# Autodesk Inventor assembly: 4-bar assembly 2
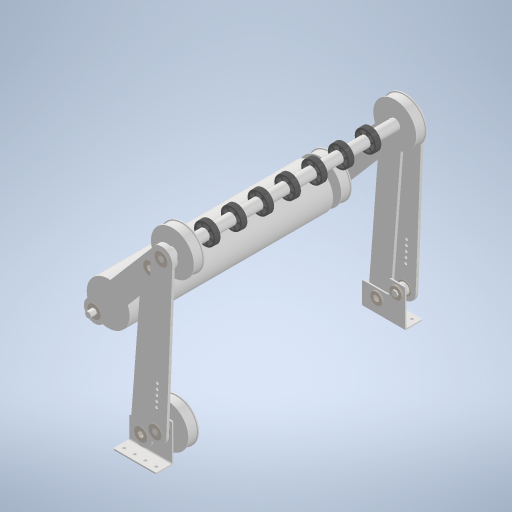
[picture p0: Inventor's stored thumbnail of the model, 512x512]
Saved by Autodesk Inventor 2023 (Build 270158030, 158C)
## iProperties
Created: 2022-07-19
Part Number: 4-bar assembly 2
Document SubType Name: Assembly
Designer: rm0990889
Author: rm0990889
## Documents named in this file (16)
- C:\Users\rm0990889\Downloads\FIRST CAD-20220720T142030Z-001\FIRST CAD\4-bar intake practice-20220720T134858Z-001\4-bar intake practice\4-bar assembly 2.iam
- C:\Users\rm0990889\Downloads\FIRST CAD-20220720T142030Z-001\FIRST CAD\4-bar intake practice-20220720T134858Z-001\4-bar intake practice\4-bar intake mount.ipt
- C:\Users\rm0990889\Downloads\FIRST CAD-20220720T142030Z-001\FIRST CAD\4-bar intake practice-20220720T134858Z-001\4-bar intake practice\4-bar intake (14.112) bar.ipt
- C:\Users\rm0990889\Downloads\FIRST CAD-20220720T142030Z-001\FIRST CAD\4-bar intake practice-20220720T134858Z-001\4-bar intake practice\am-2986 FR8ZZ Hex Bearing.ipt
- C:\Users\rm0990889\Downloads\FIRST CAD-20220720T142030Z-001\FIRST CAD\4-bar intake practice-20220720T134858Z-001\4-bar intake practice\4-bar intake spacer.ipt
- C:\Users\rm0990889\Downloads\FIRST CAD-20220720T142030Z-001\FIRST CAD\4-bar intake practice-20220720T134858Z-001\4-bar intake practice\4-bar intake (14.258) bar.ipt
- C:\Users\rm0990889\Downloads\FIRST CAD-20220720T142030Z-001\FIRST CAD\4-bar intake practice-20220720T134858Z-001\4-bar intake practice\4-bar intake (24) shaft.ipt
- C:\Users\rm0990889\Downloads\FIRST CAD-20220720T142030Z-001\FIRST CAD\4-bar intake practice-20220720T134858Z-001\4-bar intake practice\4-bar intake peg.ipt
- C:\Users\rm0990889\Downloads\FIRST CAD-20220720T142030Z-001\FIRST CAD\4-bar intake practice-20220720T134858Z-001\4-bar intake practice\4-bar intake (2) shaft.ipt
- C:\Users\rm0990889\Downloads\FIRST CAD-20220720T142030Z-001\FIRST CAD\4-bar intake practice-20220720T134858Z-001\4-bar intake practice\4-bar intake () pully.ipt
- C:\Users\rm0990889\Downloads\FIRST CAD-20220720T142030Z-001\FIRST CAD\4-bar intake practice-20220720T134858Z-001\4-bar intake practice\am-3462 2IN Molded 500Hex Compliant Wheel REV2.ipt
- C:\Users\rm0990889\Downloads\FIRST CAD-20220720T142030Z-001\FIRST CAD\4-bar intake practice-20220720T134858Z-001\4-bar intake practice\4-bar intake (2_) spacer.ipt
- C:\Users\rm0990889\Downloads\FIRST CAD-20220720T142030Z-001\FIRST CAD\4-bar intake practice-20220720T134858Z-001\4-bar intake practice\4-bar intake block.ipt
- C:\Users\rm0990889\Downloads\FIRST CAD-20220720T142030Z-001\FIRST CAD\4-bar intake practice-20220720T134858Z-001\4-bar intake practice\4-bar intake roller.ipt
- C:\Users\rm0990889\Downloads\FIRST CAD-20220720T142030Z-001\FIRST CAD\4-bar intake practice-20220720T134858Z-001\4-bar intake practice\4-bar intake (1_) spacer.ipt
- C:\Users\rm0990889\Downloads\FIRST CAD-20220720T142030Z-001\FIRST CAD\4-bar intake practice-20220720T134858Z-001\4-bar intake practice\4-bar intake mount(alt).ipt
## Components (63 placed, 15 different names)
1. 4-bar intake mount:1 — Insert:1, Insert:2, Flush:3, Flush:4
2. 4-bar intake (14.112) bar:1 — Insert:3, Insert:4
3. am-2986 FR8ZZ Hex Bearing:1 — Insert:1, Insert:5
4. am-2986 FR8ZZ Hex Bearing:2 — Insert:2, Insert:6, Insert:11
5. am-2986 FR8ZZ Hex Bearing:3 — Insert:3, Insert:5
6. am-2986 FR8ZZ Hex Bearing:4 — Insert:4, Mate:33
7. am-2986 FR8ZZ Hex Bearing:5 — Insert:8, Insert:10, Mate:7
8. am-2986 FR8ZZ Hex Bearing:6 — Insert:19, Mate:37, Mate:38, Insert:45
9. am-2986 FR8ZZ Hex Bearing:7 — Insert:9, Mate:1, Mate:2
10. am-2986 FR8ZZ Hex Bearing:8 — Insert:21, Mate:50
11. am-2986 FR8ZZ Hex Bearing:9 — Insert:20, Mate:33
12. am-2986 FR8ZZ Hex Bearing:10 — Insert:22, Mate:54, Mate:55
13. am-2986 FR8ZZ Hex Bearing:11 — Insert:24, Flush:2, Mate:51, Mate:53
14. am-2986 FR8ZZ Hex Bearing:12 — Insert:23, Mate:49
15. am-2986 FR8ZZ Hex Bearing:13 — Insert:49, Insert:56
16. am-2986 FR8ZZ Hex Bearing:14 — Insert:50, Insert:55
17. 4-bar intake spacer:2 — Mate:9, Insert:14, Mate:50
18. 4-bar intake spacer:3 — Insert:14, Mate:10, Insert:15, Insert:26
19. 4-bar intake spacer:4 — Insert:6, Insert:7
20. 4-bar intake spacer:5 — Insert:35, Insert:62
21. 4-bar intake spacer:6 — Insert:7, Insert:10
22. 4-bar intake (14.258) bar:1 — Insert:8, Insert:9, Insert:25
23. 4-bar intake (24) shaft:1 — Mate:37, Mate:38, Mate:39, Mate:40, Mate:54, Mate:55
24. 4-bar intake (24) shaft:2 — Mate:1, Mate:2, Mate:9, Mate:10, Mate:11, Mate:30, Mate:31, Mate:32, Mate:34, Mate:35, Mate:36, Mate:41, Mate:42, Mate:43, Mate:44, Mate:51, Mate:52
25. 4-bar intake peg:1 — Mate:47, Mate:48, Flush:1
26. 4-bar intake (2) shaft:2 — Mate:5, Mate:6, Mate:7
27. 4-bar intake () pully:1 — Mate:5, Mate:6, Insert:11
28. 4-bar intake () pully:2 — Insert:15, Mate:11, Insert:26, Mate:30, Mate:31, Insert:27
29. am-3462 2IN Molded 500Hex Compliant Wheel REV2:8 — Insert:34, Insert:37
30. am-3462 2IN Molded 500Hex Compliant Wheel REV2:9 — Insert:32, Insert:33
31. am-3462 2IN Molded 500Hex Compliant Wheel REV2:10 — Insert:30, Insert:31
32. am-3462 2IN Molded 500Hex Compliant Wheel REV2:11 — Insert:28, Insert:29
33. 4-bar intake block:1 — Insert:22, Insert:23, Insert:24, Insert:59
34. 4-bar intake block:2 — Insert:19, Insert:20, Insert:21, Insert:25
35. 4-bar intake (2_) spacer:8 — Insert:37, Mate:41, Insert:38
36. 4-bar intake (2_) spacer:9 — Insert:33, Mate:36, Insert:34
37. 4-bar intake (2_) spacer:11 — Insert:27, Mate:32, Insert:28
38. 4-bar intake (2_) spacer:12 — Insert:29, Mate:34, Insert:30
39. 4-bar intake (2_) spacer:13 — Insert:31, Mate:35, Insert:32
40. 4-bar intake roller:1 — Mate:39, Mate:40, Insert:35, Insert:46
41. am-3462 2IN Molded 500Hex Compliant Wheel REV2:12 — Insert:38, Insert:39
42. am-3462 2IN Molded 500Hex Compliant Wheel REV2:13 — Insert:40, Insert:41
43. am-3462 2IN Molded 500Hex Compliant Wheel REV2:15 — Insert:42, Insert:43
44. 4-bar intake (2_) spacer:15 — Insert:39, Mate:42, Insert:40
45. 4-bar intake (2_) spacer:16 — Insert:41, Mate:43, Insert:42
46. 4-bar intake (2_) spacer:17 — Insert:43, Mate:44, Insert:47
47. 4-bar intake (1_) spacer:1 — Insert:45, Insert:46
48. 4-bar intake spacer:7 — Insert:47, Insert:48
49. 4-bar intake () pully:4 — Insert:48, Insert:61
50. 4-bar intake mount(alt):1 — Insert:49, Insert:50, Flush:3, Flush:4
51. 4-bar intake (14.112) bar:2 — Insert:51, Insert:52, Insert:55
52. 4-bar intake (14.258) bar:2 — Insert:53, Insert:54, Insert:59
53. am-2986 FR8ZZ Hex Bearing:15 — Insert:52, Mate:49
54. am-2986 FR8ZZ Hex Bearing:16 — Insert:54, Insert:58, Mate:47, Mate:48, Flush:1
55. am-2986 FR8ZZ Hex Bearing:17 — Insert:51
56. am-2986 FR8ZZ Hex Bearing:18 — Insert:53, Flush:2, Mate:52
57. 4-bar intake spacer:8 — Insert:56, Insert:57
58. 4-bar intake spacer:9 — Insert:57, Insert:58
59. 4-bar intake spacer:11 — Insert:61, Mate:53
60. 4-bar intake spacer:12 — Insert:63, Insert:64
61. 4-bar intake spacer:14 — Insert:65
62. 4-bar intake spacer:15 — Insert:62, Insert:63
63. 4-bar intake () pully:5 — Insert:64, Insert:65
## Relationships (93: Insert 57, Mate 32, Flush 4)
- Insert:1: 4-bar intake mount:1 ↔ am-2986 FR8ZZ Hex Bearing:1
- Insert:2: 4-bar intake mount:1 ↔ am-2986 FR8ZZ Hex Bearing:2
- Insert:3: 4-bar intake (14.112) bar:1 ↔ am-2986 FR8ZZ Hex Bearing:3
- Insert:4: 4-bar intake (14.112) bar:1 ↔ am-2986 FR8ZZ Hex Bearing:4
- Insert:5: am-2986 FR8ZZ Hex Bearing:1 ↔ am-2986 FR8ZZ Hex Bearing:3
- Insert:6: am-2986 FR8ZZ Hex Bearing:2 ↔ 4-bar intake spacer:4
- Insert:7: 4-bar intake spacer:4 ↔ 4-bar intake spacer:6
- Insert:8: am-2986 FR8ZZ Hex Bearing:5 ↔ 4-bar intake (14.258) bar:1
- Insert:9: am-2986 FR8ZZ Hex Bearing:7 ↔ 4-bar intake (14.258) bar:1
- Insert:10: am-2986 FR8ZZ Hex Bearing:5 ↔ 4-bar intake spacer:6
- Mate:1: am-2986 FR8ZZ Hex Bearing:7 ↔ 4-bar intake (24) shaft:2
- Mate:2: am-2986 FR8ZZ Hex Bearing:7 ↔ 4-bar intake (24) shaft:2
- Mate:5: 4-bar intake (2) shaft:2 ↔ 4-bar intake () pully:1
- Mate:6: 4-bar intake (2) shaft:2 ↔ 4-bar intake () pully:1
- Insert:11: am-2986 FR8ZZ Hex Bearing:2 ↔ 4-bar intake () pully:1
- Mate:7: am-2986 FR8ZZ Hex Bearing:5 ↔ 4-bar intake (2) shaft:2
- Mate:9: 4-bar intake spacer:2 ↔ 4-bar intake (24) shaft:2
- Insert:14: 4-bar intake spacer:2 ↔ 4-bar intake spacer:3
- Mate:10: 4-bar intake spacer:3 ↔ 4-bar intake (24) shaft:2
- Insert:15: 4-bar intake spacer:3 ↔ 4-bar intake () pully:2
- Mate:11: 4-bar intake (24) shaft:2 ↔ 4-bar intake () pully:2
- Insert:19: am-2986 FR8ZZ Hex Bearing:6 ↔ 4-bar intake block:2
- Insert:20: am-2986 FR8ZZ Hex Bearing:9 ↔ 4-bar intake block:2
- Insert:21: am-2986 FR8ZZ Hex Bearing:8 ↔ 4-bar intake block:2
- Insert:22: am-2986 FR8ZZ Hex Bearing:10 ↔ 4-bar intake block:1
- Insert:23: am-2986 FR8ZZ Hex Bearing:12 ↔ 4-bar intake block:1
- Insert:24: am-2986 FR8ZZ Hex Bearing:11 ↔ 4-bar intake block:1
- Insert:25: 4-bar intake (14.258) bar:1 ↔ 4-bar intake block:2
- Insert:26: 4-bar intake spacer:3 ↔ 4-bar intake () pully:2
- Mate:30: 4-bar intake (24) shaft:2 ↔ 4-bar intake () pully:2
- Mate:31: 4-bar intake (24) shaft:2 ↔ 4-bar intake () pully:2
- Insert:27: 4-bar intake () pully:2 ↔ 4-bar intake (2_) spacer:11
- Mate:32: 4-bar intake (24) shaft:2 ↔ 4-bar intake (2_) spacer:11
- Insert:28: am-3462 2IN Molded 500Hex Compliant Wheel REV2:11 ↔ 4-bar intake (2_) spacer:11
- Mate:33: am-2986 FR8ZZ Hex Bearing:4 ↔ am-2986 FR8ZZ Hex Bearing:9
- Insert:29: am-3462 2IN Molded 500Hex Compliant Wheel REV2:11 ↔ 4-bar intake (2_) spacer:12
- Mate:34: 4-bar intake (24) shaft:2 ↔ 4-bar intake (2_) spacer:12
- Insert:30: am-3462 2IN Molded 500Hex Compliant Wheel REV2:10 ↔ 4-bar intake (2_) spacer:12
- Insert:31: am-3462 2IN Molded 500Hex Compliant Wheel REV2:10 ↔ 4-bar intake (2_) spacer:13
- Mate:35: 4-bar intake (24) shaft:2 ↔ 4-bar intake (2_) spacer:13
- Insert:32: am-3462 2IN Molded 500Hex Compliant Wheel REV2:9 ↔ 4-bar intake (2_) spacer:13
- Insert:33: am-3462 2IN Molded 500Hex Compliant Wheel REV2:9 ↔ 4-bar intake (2_) spacer:9
- Mate:36: 4-bar intake (24) shaft:2 ↔ 4-bar intake (2_) spacer:9
- Insert:34: am-3462 2IN Molded 500Hex Compliant Wheel REV2:8 ↔ 4-bar intake (2_) spacer:9
- Mate:37: am-2986 FR8ZZ Hex Bearing:6 ↔ 4-bar intake (24) shaft:1
- Mate:38: am-2986 FR8ZZ Hex Bearing:6 ↔ 4-bar intake (24) shaft:1
- Mate:39: 4-bar intake (24) shaft:1 ↔ 4-bar intake roller:1
- Mate:40: 4-bar intake (24) shaft:1 ↔ 4-bar intake roller:1
- Insert:35: 4-bar intake spacer:5 ↔ 4-bar intake roller:1
- Insert:37: am-3462 2IN Molded 500Hex Compliant Wheel REV2:8 ↔ 4-bar intake (2_) spacer:8
- Mate:41: 4-bar intake (24) shaft:2 ↔ 4-bar intake (2_) spacer:8
- Insert:38: 4-bar intake (2_) spacer:8 ↔ am-3462 2IN Molded 500Hex Compliant Wheel REV2:12
- Insert:39: am-3462 2IN Molded 500Hex Compliant Wheel REV2:12 ↔ 4-bar intake (2_) spacer:15
- Mate:42: 4-bar intake (24) shaft:2 ↔ 4-bar intake (2_) spacer:15
- Insert:40: am-3462 2IN Molded 500Hex Compliant Wheel REV2:13 ↔ 4-bar intake (2_) spacer:15
- Insert:41: am-3462 2IN Molded 500Hex Compliant Wheel REV2:13 ↔ 4-bar intake (2_) spacer:16
- Mate:43: 4-bar intake (24) shaft:2 ↔ 4-bar intake (2_) spacer:16
- Insert:42: am-3462 2IN Molded 500Hex Compliant Wheel REV2:15 ↔ 4-bar intake (2_) spacer:16
- Insert:43: am-3462 2IN Molded 500Hex Compliant Wheel REV2:15 ↔ 4-bar intake (2_) spacer:17
- Mate:44: 4-bar intake (24) shaft:2 ↔ 4-bar intake (2_) spacer:17
- Insert:45: am-2986 FR8ZZ Hex Bearing:6 ↔ 4-bar intake (1_) spacer:1
- Insert:46: 4-bar intake roller:1 ↔ 4-bar intake (1_) spacer:1
- Insert:47: 4-bar intake (2_) spacer:17 ↔ 4-bar intake spacer:7
- Insert:48: 4-bar intake spacer:7 ↔ 4-bar intake () pully:4
- Insert:49: am-2986 FR8ZZ Hex Bearing:13 ↔ 4-bar intake mount(alt):1
- Insert:50: am-2986 FR8ZZ Hex Bearing:14 ↔ 4-bar intake mount(alt):1
- Insert:51: 4-bar intake (14.112) bar:2 ↔ am-2986 FR8ZZ Hex Bearing:17
- Insert:52: 4-bar intake (14.112) bar:2 ↔ am-2986 FR8ZZ Hex Bearing:15
- Insert:53: 4-bar intake (14.258) bar:2 ↔ am-2986 FR8ZZ Hex Bearing:18
- Insert:54: 4-bar intake (14.258) bar:2 ↔ am-2986 FR8ZZ Hex Bearing:16
- Insert:55: am-2986 FR8ZZ Hex Bearing:14 ↔ 4-bar intake (14.112) bar:2
- Insert:56: am-2986 FR8ZZ Hex Bearing:13 ↔ 4-bar intake spacer:8
- Insert:57: 4-bar intake spacer:8 ↔ 4-bar intake spacer:9
- Insert:58: am-2986 FR8ZZ Hex Bearing:16 ↔ 4-bar intake spacer:9
- Mate:47: 4-bar intake peg:1 ↔ am-2986 FR8ZZ Hex Bearing:16
- Mate:48: 4-bar intake peg:1 ↔ am-2986 FR8ZZ Hex Bearing:16
- Flush:1: 4-bar intake peg:1 ↔ am-2986 FR8ZZ Hex Bearing:16
- Insert:59: 4-bar intake block:1 ↔ 4-bar intake (14.258) bar:2
- Mate:49: am-2986 FR8ZZ Hex Bearing:12 ↔ am-2986 FR8ZZ Hex Bearing:15
- Insert:61: 4-bar intake () pully:4 ↔ 4-bar intake spacer:11
- Mate:50: am-2986 FR8ZZ Hex Bearing:8 ↔ 4-bar intake spacer:2
- Insert:62: 4-bar intake spacer:5 ↔ 4-bar intake spacer:15
- Insert:63: 4-bar intake spacer:12 ↔ 4-bar intake spacer:15
- Insert:64: 4-bar intake spacer:12 ↔ 4-bar intake () pully:5
- Insert:65: 4-bar intake spacer:14 ↔ 4-bar intake () pully:5
- Flush:2: am-2986 FR8ZZ Hex Bearing:11 ↔ am-2986 FR8ZZ Hex Bearing:18
- Mate:51: am-2986 FR8ZZ Hex Bearing:11 ↔ 4-bar intake (24) shaft:2
- Mate:52: 4-bar intake (24) shaft:2 ↔ am-2986 FR8ZZ Hex Bearing:18
- Mate:53: am-2986 FR8ZZ Hex Bearing:11 ↔ 4-bar intake spacer:11
- Mate:54: am-2986 FR8ZZ Hex Bearing:10 ↔ 4-bar intake (24) shaft:1
- Mate:55: am-2986 FR8ZZ Hex Bearing:10 ↔ 4-bar intake (24) shaft:1
- Flush:3: 4-bar intake mount:1 ↔ 4-bar intake mount(alt):1
- Flush:4: 4-bar intake mount:1 ↔ 4-bar intake mount(alt):1
